# Autodesk Inventor assembly: КВ33.044.500 - Каретка оси Y
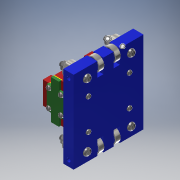
[picture p0: Inventor's stored thumbnail of the model, 180x180]
Saved by Autodesk Inventor 2019 (Build 230136000, 136)
## iProperties
Created: 2019-07-21
Part Number: КВ33.044.500 - Каретка оси Y
Material: Типовые
Document SubType Name: Assembly
Designer: Петров Иван
Author: Петров Иван
## Documents named in this file (11)
- E:\IVAN\Kvantoriada2019\optimal_gripper\hardware\КВ33.044.500 - Каретка оси Y.iam
- E:\IVAN\Kvantoriada2019\optimal_gripper\hardware\КВ33.044.501 - Каретка оси Y.ipt
- E:\IVAN\Kvantoriada2019\optimal_gripper\hardware\Стандартные изделия\Подшипник 624Z.ipt
- E:\IVAN\Kvantoriada2019\optimal_gripper\hardware\КВ33.044.502 - Фиксатор оси Y.ipt
- E:\IVAN\Kvantoriada2019\optimal_gripper\hardware\КВ33.044.503 - Прижим ремня.ipt
- C:\Users\Петров Иван\Documents\Inventor\Content Center Files\R2019\ru-RU\AS 1427(10)\AS 1427 - M3,5 x 45(7).ipt
- C:\Users\Петров Иван\Documents\Inventor\Content Center Files\R2019\ru-RU\CNS 9671\CNS 9671 - M4 x 25.ipt
- C:\Users\Петров Иван\Documents\Inventor\Content Center Files\R2019\ru-RU\CNS 9671\CNS 9671 - M2,6 x 18.ipt
- C:\Users\Петров Иван\Documents\Inventor\Content Center Files\R2019\ru-RU\CNS 9671\CNS 9671 - M2,6 x 6.ipt
- C:\Users\Петров Иван\Documents\Inventor\Content Center Files\R2019\ru-RU\AS 1237 (2.1)\AS 1237 - 4.ipt
- C:\Users\Петров Иван\Documents\Inventor\Content Center Files\R2019\ru-RU\ANSI B18.2.4.2M\ANSI B18.2.4.2M - M4x0,7 - 7.ipt
## Components (52 placed, 10 different names)
1. КВ33.044.501 - Каретка оси Y:1 — Совмещение:1, Совмещение:2, Совмещение:3, Совмещение:4, Совмещение:5, Совмещение:6, 2.5, Совмещение:8, Совмещение:9, Совмещение:10, Совмещение:11, Совмещение:12, Совмещение:13, Совмещение:14, Совмещение:15, Совмещение:16, Совмещение:17, Совмещение:18, Совмещение:19, Совмещение:20, Совмещение:21, Совмещение:22, Совмещение:27, Совмещение:28, Совмещение:29, Совмещение:30, Вставка:1, Вставка:2, Вставка:3, Вставка:4, Вставка:5, Вставка:6, Вставка:7, Вставка:8, Совмещение:32, Вставка:20, Вставка:21, Вставка:22, Вставка:23
2. Подшипник 624Z:1 — Совмещение:1, Совмещение:8, Вставка:32
3. Подшипник 624Z:2 — Совмещение:4, Совмещение:5, Вставка:29
4. Подшипник 624Z:3 — Совмещение:3, Совмещение:6, Вставка:19
5. Подшипник 624Z:4 — Совмещение:2, 2.5, Вставка:26
6. Подшипник 624Z:5 — Совмещение:9, Совмещение:15
7. Подшипник 624Z:6 — Совмещение:10, Совмещение:16
8. Подшипник 624Z:7 — Совмещение:11, Совмещение:13
9. Подшипник 624Z:8 — Совмещение:12, Совмещение:14
10. КВ33.044.502 - Фиксатор оси Y:1 — Совмещение:17, Совмещение:18, Совмещение:19, Совмещение:23, Заподлицо:1, Совмещение:24
11. КВ33.044.502 - Фиксатор оси Y:2 — Совмещение:20, Совмещение:21, Совмещение:22, Совмещение:25, Заподлицо:2, Совмещение:26
12. КВ33.044.503 - Прижим ремня:1 — Совмещение:25, Заподлицо:2, Совмещение:26, Вставка:13, Вставка:14, Вставка:15, Вставка:16
13. КВ33.044.503 - Прижим ремня:2 — Совмещение:23, Заподлицо:1, Совмещение:24, Вставка:9, Вставка:10, Вставка:11, Вставка:12
14. AS 1427 (8) - метрическая M3,5 x 45:1 — Совмещение:27, Совмещение:28
15. AS 1427 (8) - метрическая M3,5 x 45:2 — Совмещение:29, Совмещение:30
16. CNS 9671 M4 x 25:1 — Вставка:1
17. CNS 9671 M4 x 25:2 — Вставка:2
18. CNS 9671 M4 x 25:3 — Вставка:3, Совмещение:31
19. CNS 9671 M4 x 25:4 — Вставка:4
20. CNS 9671 M2,6 x 18:1 — Вставка:5
21. CNS 9671 M2,6 x 18:2 — Вставка:6
22. CNS 9671 M2,6 x 18:3 — Вставка:7
23. CNS 9671 M2,6 x 18:4 — Вставка:8
24. CNS 9671 M2,6 x 6:1 — Вставка:9
25. CNS 9671 M2,6 x 6:2 — Вставка:10
26. CNS 9671 M2,6 x 6:3 — Вставка:11
27. CNS 9671 M2,6 x 6:4 — Вставка:12
28. CNS 9671 M2,6 x 6:5 — Вставка:13
29. CNS 9671 M2,6 x 6:6 — Вставка:14
30. CNS 9671 M2,6 x 6:7 — Вставка:15
31. CNS 9671 M2,6 x 6:8 — Вставка:16
32. AS 1237 (2.1) 4:1 — Совмещение:31, Совмещение:32, Вставка:17
33. AS 1237 (2.1) 4:2 — Вставка:17, Вставка:18
34. AS 1237 (2.1) 4:3 — Вставка:18
35. AS 1237 (2.1) 4:4 — Вставка:19, Вставка:33
36. AS 1237 (2.1) 4:5 — Вставка:20, Вставка:24
37. AS 1237 (2.1) 4:6 — Вставка:21
38. AS 1237 (2.1) 4:7 — Вставка:22, Вставка:30
39. AS 1237 (2.1) 4:8 — Вставка:23, Вставка:27
40. AS 1237 (2.1) 4:9 — Вставка:24, Вставка:25
41. AS 1237 (2.1) 4:10 — Вставка:25
42. AS 1237 (2.1) 4:11 — Вставка:26, Вставка:34
43. AS 1237 (2.1) 4:12 — Вставка:27, Вставка:28
44. AS 1237 (2.1) 4:13 — Вставка:28
45. AS 1237 (2.1) 4:14 — Вставка:29, Вставка:35
46. AS 1237 (2.1) 4:15 — Вставка:30, Вставка:31
47. AS 1237 (2.1) 4:16 — Вставка:31
48. AS 1237 (2.1) 4:17 — Вставка:32, Вставка:36
49. ANSI B18.2.4.2M M4x0,7:1 — Вставка:33
50. ANSI B18.2.4.2M M4x0,7:2 — Вставка:34
51. ANSI B18.2.4.2M M4x0,7:3 — Вставка:35
52. ANSI B18.2.4.2M M4x0,7:4 — Вставка:36
## Relationships (70: Insert 36, Mate 32, Flush 2)
- Совмещение:1 [Mate]: КВ33.044.501 - Каретка оси Y:1 ↔ Подшипник 624Z:1
- Совмещение:2 [Mate]: КВ33.044.501 - Каретка оси Y:1 ↔ Подшипник 624Z:4
- Совмещение:3 [Mate]: КВ33.044.501 - Каретка оси Y:1 ↔ Подшипник 624Z:3
- Совмещение:4 [Mate]: КВ33.044.501 - Каретка оси Y:1 ↔ Подшипник 624Z:2
- Совмещение:5 [Mate] (2.5 mm): КВ33.044.501 - Каретка оси Y:1 ↔ Подшипник 624Z:2
- Совмещение:6 [Mate] (2.5 mm): КВ33.044.501 - Каретка оси Y:1 ↔ Подшипник 624Z:3
- 2.5 [Mate] (2.5 mm): КВ33.044.501 - Каретка оси Y:1 ↔ Подшипник 624Z:4
- Совмещение:8 [Mate] (2.5 mm): КВ33.044.501 - Каретка оси Y:1 ↔ Подшипник 624Z:1
- Совмещение:9 [Mate]: КВ33.044.501 - Каретка оси Y:1 ↔ Подшипник 624Z:5
- Совмещение:10 [Mate]: КВ33.044.501 - Каретка оси Y:1 ↔ Подшипник 624Z:6
- Совмещение:11 [Mate]: КВ33.044.501 - Каретка оси Y:1 ↔ Подшипник 624Z:7
- Совмещение:12 [Mate]: КВ33.044.501 - Каретка оси Y:1 ↔ Подшипник 624Z:8
- Совмещение:13 [Mate] (0.5 mm): КВ33.044.501 - Каретка оси Y:1 ↔ Подшипник 624Z:7
- Совмещение:14 [Mate] (0.5 mm): КВ33.044.501 - Каретка оси Y:1 ↔ Подшипник 624Z:8
- Совмещение:15 [Mate] (0.5 mm): КВ33.044.501 - Каретка оси Y:1 ↔ Подшипник 624Z:5
- Совмещение:16 [Mate] (0.5 mm): КВ33.044.501 - Каретка оси Y:1 ↔ Подшипник 624Z:6
- Совмещение:17 [Mate]: КВ33.044.501 - Каретка оси Y:1 ↔ КВ33.044.502 - Фиксатор оси Y:1
- Совмещение:18 [Mate]: КВ33.044.501 - Каретка оси Y:1 ↔ КВ33.044.502 - Фиксатор оси Y:1
- Совмещение:19 [Mate]: КВ33.044.501 - Каретка оси Y:1 ↔ КВ33.044.502 - Фиксатор оси Y:1
- Совмещение:20 [Mate]: КВ33.044.501 - Каретка оси Y:1 ↔ КВ33.044.502 - Фиксатор оси Y:2
- Совмещение:21 [Mate]: КВ33.044.501 - Каретка оси Y:1 ↔ КВ33.044.502 - Фиксатор оси Y:2
- Совмещение:22 [Mate]: КВ33.044.501 - Каретка оси Y:1 ↔ КВ33.044.502 - Фиксатор оси Y:2
- Совмещение:23 [Mate]: КВ33.044.502 - Фиксатор оси Y:1 ↔ КВ33.044.503 - Прижим ремня:2
- Заподлицо:1 [Flush]: КВ33.044.502 - Фиксатор оси Y:1 ↔ КВ33.044.503 - Прижим ремня:2
- Совмещение:24 [Mate]: КВ33.044.502 - Фиксатор оси Y:1 ↔ КВ33.044.503 - Прижим ремня:2
- Совмещение:25 [Mate]: КВ33.044.502 - Фиксатор оси Y:2 ↔ КВ33.044.503 - Прижим ремня:1
- Заподлицо:2 [Flush]: КВ33.044.502 - Фиксатор оси Y:2 ↔ КВ33.044.503 - Прижим ремня:1
- Совмещение:26 [Mate]: КВ33.044.502 - Фиксатор оси Y:2 ↔ КВ33.044.503 - Прижим ремня:1
- Совмещение:27 [Mate]: КВ33.044.501 - Каретка оси Y:1 ↔ AS 1427 (8) - метрическая M3,5 x 45:1
- Совмещение:28 [Mate]: КВ33.044.501 - Каретка оси Y:1 ↔ AS 1427 (8) - метрическая M3,5 x 45:1
- Совмещение:29 [Mate]: КВ33.044.501 - Каретка оси Y:1 ↔ AS 1427 (8) - метрическая M3,5 x 45:2
- Совмещение:30 [Mate]: КВ33.044.501 - Каретка оси Y:1 ↔ AS 1427 (8) - метрическая M3,5 x 45:2
- Вставка:1 [Insert]: КВ33.044.501 - Каретка оси Y:1 ↔ CNS 9671 M4 x 25:1
- Вставка:2 [Insert]: КВ33.044.501 - Каретка оси Y:1 ↔ CNS 9671 M4 x 25:2
- Вставка:3 [Insert]: КВ33.044.501 - Каретка оси Y:1 ↔ CNS 9671 M4 x 25:3
- Вставка:4 [Insert]: КВ33.044.501 - Каретка оси Y:1 ↔ CNS 9671 M4 x 25:4
- Вставка:5 [Insert]: КВ33.044.501 - Каретка оси Y:1 ↔ CNS 9671 M2,6 x 18:1
- Вставка:6 [Insert]: КВ33.044.501 - Каретка оси Y:1 ↔ CNS 9671 M2,6 x 18:2
- Вставка:7 [Insert]: КВ33.044.501 - Каретка оси Y:1 ↔ CNS 9671 M2,6 x 18:3
- Вставка:8 [Insert]: КВ33.044.501 - Каретка оси Y:1 ↔ CNS 9671 M2,6 x 18:4
- Вставка:9 [Insert]: КВ33.044.503 - Прижим ремня:2 ↔ CNS 9671 M2,6 x 6:1
- Вставка:10 [Insert]: КВ33.044.503 - Прижим ремня:2 ↔ CNS 9671 M2,6 x 6:2
- Вставка:11 [Insert]: КВ33.044.503 - Прижим ремня:2 ↔ CNS 9671 M2,6 x 6:3
- Вставка:12 [Insert]: КВ33.044.503 - Прижим ремня:2 ↔ CNS 9671 M2,6 x 6:4
- Вставка:13 [Insert]: КВ33.044.503 - Прижим ремня:1 ↔ CNS 9671 M2,6 x 6:5
- Вставка:14 [Insert]: КВ33.044.503 - Прижим ремня:1 ↔ CNS 9671 M2,6 x 6:6
- Вставка:15 [Insert]: КВ33.044.503 - Прижим ремня:1 ↔ CNS 9671 M2,6 x 6:7
- Вставка:16 [Insert]: КВ33.044.503 - Прижим ремня:1 ↔ CNS 9671 M2,6 x 6:8
- Совмещение:31 [Mate]: CNS 9671 M4 x 25:3 ↔ AS 1237 (2.1) 4:1
- Совмещение:32 [Mate]: КВ33.044.501 - Каретка оси Y:1 ↔ AS 1237 (2.1) 4:1
- Вставка:17 [Insert]: AS 1237 (2.1) 4:1 ↔ AS 1237 (2.1) 4:2
- Вставка:18 [Insert]: AS 1237 (2.1) 4:2 ↔ AS 1237 (2.1) 4:3
- Вставка:19 [Insert]: Подшипник 624Z:3 ↔ AS 1237 (2.1) 4:4
- Вставка:20 [Insert]: КВ33.044.501 - Каретка оси Y:1 ↔ AS 1237 (2.1) 4:5
- Вставка:21 [Insert]: КВ33.044.501 - Каретка оси Y:1 ↔ AS 1237 (2.1) 4:6
- Вставка:22 [Insert]: КВ33.044.501 - Каретка оси Y:1 ↔ AS 1237 (2.1) 4:7
- Вставка:23 [Insert]: КВ33.044.501 - Каретка оси Y:1 ↔ AS 1237 (2.1) 4:8
- Вставка:24 [Insert]: AS 1237 (2.1) 4:5 ↔ AS 1237 (2.1) 4:9
- Вставка:25 [Insert]: AS 1237 (2.1) 4:9 ↔ AS 1237 (2.1) 4:10
- Вставка:26 [Insert]: Подшипник 624Z:4 ↔ AS 1237 (2.1) 4:11
- Вставка:27 [Insert]: AS 1237 (2.1) 4:8 ↔ AS 1237 (2.1) 4:12
- Вставка:28 [Insert]: AS 1237 (2.1) 4:12 ↔ AS 1237 (2.1) 4:13
- Вставка:29 [Insert]: Подшипник 624Z:2 ↔ AS 1237 (2.1) 4:14
- Вставка:30 [Insert]: AS 1237 (2.1) 4:7 ↔ AS 1237 (2.1) 4:15
- Вставка:31 [Insert]: AS 1237 (2.1) 4:15 ↔ AS 1237 (2.1) 4:16
- Вставка:32 [Insert]: Подшипник 624Z:1 ↔ AS 1237 (2.1) 4:17
- Вставка:33 [Insert]: AS 1237 (2.1) 4:4 ↔ ANSI B18.2.4.2M M4x0,7:1
- Вставка:34 [Insert]: AS 1237 (2.1) 4:11 ↔ ANSI B18.2.4.2M M4x0,7:2
- Вставка:35 [Insert]: AS 1237 (2.1) 4:14 ↔ ANSI B18.2.4.2M M4x0,7:3
- Вставка:36 [Insert]: AS 1237 (2.1) 4:17 ↔ ANSI B18.2.4.2M M4x0,7:4
